# Autodesk Inventor assembly: trzymak
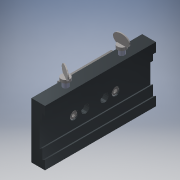
[picture p0: Inventor's stored thumbnail of the model, 180x180]
Saved by Autodesk Inventor 2019 (Build 230136000, 136)
## iProperties
Created: 2020-08-30
Part Number: trzymak
Document SubType Name: Assembly
Designer: estee
Author: estee
## Documents named in this file (7)
- C:\Users\estee\OneDrive\Pulpit\estere\1\MUM\najnowszyGIT\Mechanika\Moduł obrotu RET Estera\projejt\projejt\trzymak.iam
- C:\Users\estee\OneDrive\Pulpit\estere\1\MUM\najnowszyGIT\Mechanika\Moduł obrotu RET Estera\projejt\projejt\plytkaadaptacyjna.ipt
- C:\Users\estee\OneDrive\Pulpit\estere\1\MUM\najnowszyGIT\Mechanika\Moduł obrotu RET Estera\projejt\projejt\uchwytDoSzyny.iam
- C:\Users\estee\OneDrive\Pulpit\estere\1\MUM\najnowszyGIT\Mechanika\Moduł obrotu RET Estera\projejt\projejt\kolnierz.ipt
- C:\Users\estee\OneDrive\Dokumenty\Inventor\Content Center Files\R2019\en-US\ISO 4762(2)\ISO 4762 - M3 x 5ISO.ipt
- C:\Users\estee\OneDrive\Dokumenty\Inventor\Content Center Files\R2019\en-US\ISO 4762(2)\ISO 4762 - M8 x 20ISO.ipt
- C:\Users\estee\OneDrive\Dokumenty\Inventor\Content Center Files\R2019\en-US\ISO 4032(2)\ISO 4032 - M8 - ISO.ipt
## Components (11 placed, 6 different names)
1. plytkaadaptacyjna:1 — Mate:1, Mate:2, Mate:3, Mate:4, Mate:5, Mate:6, Mate:7, Mate:8, Mate:9, Mate:10, Mate:11, Mate:12, Mate:13, Mate:14, Mate:19, Mate:20
2. uchwytDoSzyny:1 [sub-assembly] — Mate:12, Mate:13, Mate:14, Mate:15, Mate:16, Mate:17, Mate:18
3. kolnierz:2 — Mate:1, Mate:2, Mate:3
4. ISO 4762 M3 x 5:1 — Mate:4, Mate:8
5. ISO 4762 M3 x 5:2 — Mate:5, Mate:11
6. ISO 4762 M3 x 5:3 — Mate:6, Mate:10
7. ISO 4762 M3 x 5:4 — Mate:7, Mate:9
8. ISO 4762 M8 x 20:1 — Mate:17, Mate:18, Mate:22
9. ISO 4762 M8 x 20:2 — Mate:15, Mate:16, Mate:21
10. ISO 4032 M8:1 — Mate:19, Mate:22
11. ISO 4032 M8:2 — Mate:20, Mate:21
## Relationships (22: Mate 22)
- Mate:1: plytkaadaptacyjna:1 ↔ kolnierz:2
- Mate:2: plytkaadaptacyjna:1 ↔ kolnierz:2
- Mate:3: plytkaadaptacyjna:1 ↔ kolnierz:2
- Mate:4: plytkaadaptacyjna:1 ↔ ISO 4762 M3 x 5:1
- Mate:5: plytkaadaptacyjna:1 ↔ ISO 4762 M3 x 5:2
- Mate:6: plytkaadaptacyjna:1 ↔ ISO 4762 M3 x 5:3
- Mate:7: plytkaadaptacyjna:1 ↔ ISO 4762 M3 x 5:4
- Mate:8: plytkaadaptacyjna:1 ↔ ISO 4762 M3 x 5:1
- Mate:9: plytkaadaptacyjna:1 ↔ ISO 4762 M3 x 5:4
- Mate:10: plytkaadaptacyjna:1 ↔ ISO 4762 M3 x 5:3
- Mate:11: plytkaadaptacyjna:1 ↔ ISO 4762 M3 x 5:2
- Mate:12: plytkaadaptacyjna:1 ↔ uchwytDoSzyny:1
- Mate:13: plytkaadaptacyjna:1 ↔ uchwytDoSzyny:1
- Mate:14: plytkaadaptacyjna:1 ↔ uchwytDoSzyny:1
- Mate:15: uchwytDoSzyny:1 ↔ ISO 4762 M8 x 20:2
- Mate:16: uchwytDoSzyny:1 ↔ ISO 4762 M8 x 20:2
- Mate:17: uchwytDoSzyny:1 ↔ ISO 4762 M8 x 20:1
- Mate:18: uchwytDoSzyny:1 ↔ ISO 4762 M8 x 20:1
- Mate:19: plytkaadaptacyjna:1 ↔ ISO 4032 M8:1
- Mate:20: plytkaadaptacyjna:1 ↔ ISO 4032 M8:2
- Mate:21: ISO 4762 M8 x 20:2 ↔ ISO 4032 M8:2
- Mate:22: ISO 4762 M8 x 20:1 ↔ ISO 4032 M8:1
